# Autodesk Inventor assembly: tendeur_complet
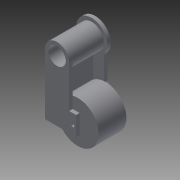
[picture p0: Inventor's stored thumbnail of the model, 180x180]
Saved by Autodesk Inventor 2014 SP1 (Build 180222100, 222)
## iProperties
Created: 2015-09-12
Part Number: tendeur_complet
Document SubType Name: Assembly
Designer: astralien3000
Author: astralien3000
## Documents named in this file (3)
- C:\Users\astralien3000\Desktop\ceres\meca\v2016\tendeur_complet.iam
- C:\Users\astralien3000\Desktop\ceres\meca\v2016\tendeur.ipt
- C:\Users\astralien3000\Desktop\ceres\meca\v2016\tendeur_roue.ipt
## Components (2 placed, 2 different names)
1. tendeur:1 — Placage:1, Placage:2
2. tendeur_roue:1 — Placage:1, Placage:2
## Relationships (2: Mate 2)
- Placage:1 [Mate]: tendeur:1 ↔ tendeur_roue:1
- Placage:2 [Mate] (0.5 mm): tendeur:1 ↔ tendeur_roue:1
